# Autodesk Inventor assembly: Z
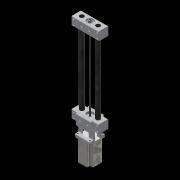
[picture p0: Inventor's stored thumbnail of the model, 180x180]
Saved by Autodesk Inventor 2016 (Build 200138000, 138)
## iProperties
Created: 2017-07-13
Part Number: Z
Document SubType Name: Assembly
Designer: ludwi
Author: ludwi
## Documents named in this file (8)
- H:\MARQ\3D\AXIS_DEV_EDT_V3\Z.iam
- H:\MARQ\3D\AXIS_DEV_EDT_V3\AXB.ipt
- H:\MARQ\3D\AXIS_DEV_EDT_V3\TuboEstructuraC.ipt
- C:\Users\ludwi\OneDrive\Documentos\Inventor\Content Center Files\R2016\en-US\DIN BEARING(1)\DIN 625 SKF - SKF 626.ipt
- H:\MARQ\3D\AXIS_DEV_EDT_V3\M6SS.ipt
- C:\Users\ludwi\OneDrive\Documentos\Inventor\Content Center Files\R2016\en-US\DIN 935\DIN 935 T1 - M6 x 1 x 10.ipt
- H:\MARQ\3D\AXIS_DEV_EDT_V3\NEMA23.ipt
- H:\MARQ\3D\AXIS_DEV_EDT_V3\MSUP.ipt
## Components (14 placed, 7 different names)
1. AXB:1 — Insert:1, Insert:2, Insert:5, Insert:6, Insert:9, Mate:2
2. AXB:2 — Insert:7, Insert:8
3. AXB:3 — Insert:3, Insert:4, Insert:7, Insert:8, Insert:10
4. AXB:4 — Insert:5, Insert:6, Insert:12, Insert:15
5. TuboEstructuraC:1 — Insert:1, Insert:3
6. TuboEstructuraC:2 — Insert:2, Insert:4
7. DIN 625 SKF SKF 626:1 — Insert:9, Mate:6
8. DIN 625 SKF SKF 626:2 — Insert:10, Mate:1, Mate:4
9. M6SS:1 — Mate:1, Mate:2, Mate:3, Mate:5, Flush:1, Insert:11
10. DIN 935 M6:1 — Mate:3, Mate:4, Flush:1
11. DIN 935 M6:2 — Mate:5, Mate:6
12. NEMA23:1 — Insert:11, Flush:2, Insert:13, Insert:14
13. MSUP:1 — Flush:2
14. MSUP:2 — Insert:12, Insert:13, Insert:14, Insert:15
## Relationships (23: Insert 15, Mate 6, Flush 2)
- Insert:1: AXB:1 ↔ TuboEstructuraC:1
- Insert:2: AXB:1 ↔ TuboEstructuraC:2
- Insert:3: AXB:3 ↔ TuboEstructuraC:1
- Insert:4: AXB:3 ↔ TuboEstructuraC:2
- Insert:5: AXB:1 ↔ AXB:4
- Insert:6: AXB:1 ↔ AXB:4
- Insert:7: AXB:2 ↔ AXB:3
- Insert:8: AXB:2 ↔ AXB:3
- Insert:9: AXB:1 ↔ DIN 625 SKF SKF 626:1
- Insert:10: AXB:3 ↔ DIN 625 SKF SKF 626:2
- Mate:1: DIN 625 SKF SKF 626:2 ↔ M6SS:1
- Mate:2: AXB:1 ↔ M6SS:1
- Mate:3: M6SS:1 ↔ DIN 935 M6:1
- Mate:4: DIN 625 SKF SKF 626:2 ↔ DIN 935 M6:1
- Mate:5: M6SS:1 ↔ DIN 935 M6:2
- Mate:6: DIN 625 SKF SKF 626:1 ↔ DIN 935 M6:2
- Flush:1: M6SS:1 ↔ DIN 935 M6:1
- Insert:11: M6SS:1 ↔ NEMA23:1
- Flush:2: NEMA23:1 ↔ MSUP:1
- Insert:12: AXB:4 ↔ MSUP:2
- Insert:13: NEMA23:1 ↔ MSUP:2
- Insert:14: NEMA23:1 ↔ MSUP:2
- Insert:15: AXB:4 ↔ MSUP:2
